# Autodesk Inventor assembly: BaseMini
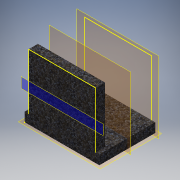
[picture p0: Inventor's stored thumbnail of the model, 180x180]
Saved by Autodesk Inventor 2016 (Build 200138000, 138)
## iProperties
Created: 2015-08-01
Part Number: BaseMini
Document SubType Name: Assembly
Designer: myhome
Author: myhome
## Documents named in this file (2)
- C:\Users\myhome\Documents\Inventor\Printer\EpoxyGraniteBase\BaseMini.iam
- C:\Users\myhome\Documents\Inventor\Printer\EpoxyGraniteBase\BaseMini.ipt
## Components (1 placed, 1 different names)
1. BaseMini:1 — Flush:1, Flush:2, Flush:3
## Relationships (3: Flush 3)
- Flush:1: BaseMini:1
- Flush:2: BaseMini:1
- Flush:3: BaseMini:1
